# Autodesk Inventor assembly: Mechanism pulso
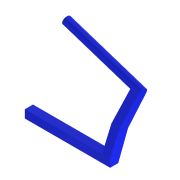
[picture p0: Inventor's stored thumbnail of the model, 180x180]
Saved by Autodesk Inventor 2020 (Build 240168000, 168)
## iProperties
Created: 2021-05-10
Part Number: Mechanism pulso
Document SubType Name: Assembly
Designer: deox
Author: deox
## Documents named in this file (3)
- C:\Users\deox\Documents\Inventor Files\Projeto Punho\Mechanism pulso.iam
- C:\Users\deox\Documents\Inventor Files\Projeto Punho\Radius_Bone1_Joint_LOWER.ipt
- C:\Users\deox\Documents\Inventor Files\Projeto Punho\Radius_Bone1_Joint_UPPER.ipt
## Components (2 placed, 2 different names)
1. Radius_Bone1_Joint_LOWER:1 — Mate:1, Flush:2
2. Radius_Bone1_Joint_UPPER:1 — Mate:1, Flush:2
## Relationships (2: Mate 1, Flush 1)
- Mate:1: Radius_Bone1_Joint_LOWER:1 ↔ Radius_Bone1_Joint_UPPER:1
- Flush:2: Radius_Bone1_Joint_LOWER:1 ↔ Radius_Bone1_Joint_UPPER:1
